# Autodesk Inventor assembly: Front_Panel_Assembly
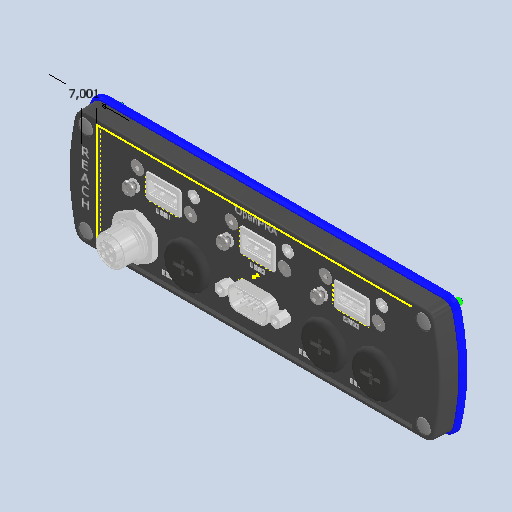
[picture p0: Inventor's stored thumbnail of the model, 512x512]
Saved by Autodesk Inventor 2022 (Build 260153000, 153)
## iProperties
Created: 2020-07-14
Part Number: Front_Panel_Assembly
Document SubType Name: Assembly
Designer: CASE-SMALL2
Author: CASE-SMALL2
## Documents named in this file (14)
- C:\Users\Viktor\Google Drive\Unicorn 2020\CAD_V2\Front_Panel\Front_Panel_Assembly.iam
- C:\Users\Viktor\Google Drive\Unicorn 2020\CAD_V2\Front_Panel\Panel\Front_Panel_Base_Assembly.iam
- C:\Users\Viktor\Google Drive\Unicorn 2020\CAD_V2\Front_Panel\Connectors\T4171110005-001\t4171110005-001.ipt
- C:\Users\Viktor\Google Drive\Unicorn 2020\CAD_V2\Front_Panel\Connectors\T4171110005-001\M12_NUT.ipt
- C:\Users\Viktor\Google Drive\Unicorn 2020\CAD_V2\Front_Panel\Connectors\MDBR-E09PM-JN0.ipt
- C:\Users\Viktor\Google Drive\Unicorn 2020\CAD_V2\Front_Panel\Connectors\MUSBR-3193-M0.ipt
- C:\Users\Viktor\Google Drive\Unicorn 2020\CAD_V2\Front_Panel\Connectors\MHDRA511M0.ipt
- C:\Users\Viktor\Google Drive\Unicorn 2020\CAD_V2\Front_Panel\Other\pop_PSZROX-0315.ipt
- C:\Users\Viktor\Google Drive\Unicorn 2020\CAD_V2\Front_Panel\Other\PG9x6mm_Plug.ipt
- C:\Users\Viktor\Google Drive\Unicorn 2020\CAD_V2\Front_Panel\Other\PG9x2.85mm_Nut.ipt
- C:\Users\Viktor\Google Drive\Unicorn 2020\CAD_V2\Front_Panel\Other\5207953-3.ipt
- C:\Users\Viktor\Google Drive\Unicorn 2020\CAD_V2\Front_Panel\Screws\ISO 4762 - M3 x 4ISO.ipt
- C:\Users\Viktor\Google Drive\Unicorn 2020\CAD_V2\Front_Panel\Screws\ISO 10642 - M3x6.ipt
- C:\Users\Viktor\Google Drive\Unicorn 2020\CAD_V2\Front_Panel\Screws\ISO 7380-1 - M3 x 8.ipt
## Components (37 placed, 13 different names)
1. Front_Pane_Basel_Assembly:1 [sub-assembly] — Rigid:1, Rigid:3, Rigid:7, Rigid:11, Rigid:17, Rigid:25, Rigid:36, Rigid:37, Rigid:38, Rigid:39, Rigid:42, Rigid:43, Rigid:45, Rigid:48, Rigid:47, Insert:1, Rigid:49, Rigid:50, Rigid:51, Rigid:52, Rigid:53, Rigid:54, Rigid:55, Rigid:56, Rigid:57, Rigid:58
2. t4171110005-001:1 — Rigid:45
3. M12_NUT:1 — Rigid:11
4. MDBR-E09PM-JN0:1 — Rigid:7
5. MUSBR-3193-M0:1 — Rigid:39
6. MUSBR-3193-M0:2 — Rigid:49
7. MUSBR-3193-M0:3 — Rigid:42, Rigid:44
8. MHDRA511M0:1 — Rigid:44
9. pop_PSZROX-0315:1 — Rigid:21, Rigid:32, Rigid:56
10. pop_PSZROX-0315:2 — Rigid:17, Rigid:20
11. pop_PSZROX-0315:3 — Rigid:22, Rigid:33, Rigid:55
12. pop_PSZROX-0315:4 — Rigid:23, Rigid:43
13. pop_PSZROX-0315:5 — Rigid:58, Rigid:59, Rigid:61
14. pop_PSZROX-0315:6 — Rigid:57, Rigid:60
15. PG9x6mm_Plug:1 — Rigid:1
16. PG9x6mm_Plug:2 — Insert:1, Angle:1
17. PG9x6mm_Plug:3 — Rigid:3, Angle:1
18. PG9x2.85mm_Nut:1 — Rigid:36
19. PG9x2.85mm_Nut:2 — Rigid:37
20. PG9x2.85mm_Nut:3 — Rigid:38
21. 5207953-3:1 — Rigid:48
22. 5207953-3:2 — Rigid:47
23. ISO 4762 - M3 x 4ISO:1 — Rigid:20
24. ISO 4762 - M3 x 4ISO:2 — Rigid:21
25. ISO 4762 - M3 x 4ISO:3 — Rigid:22
26. ISO 4762 - M3 x 4ISO:4 — Rigid:23
27. ISO 4762 - M3 x 4ISO:5 — Rigid:60
28. ISO 4762 - M3 x 4ISO:6 — Rigid:61
29. ISO 7380-1 - M3 x 8:3 — Rigid:32
30. ISO 7380-1 - M3 x 8:4 — Rigid:33
31. ISO 7380-1 - M3 x 8:5 — Rigid:59
32. ISO 10642 - M3x6:1 — Rigid:50
33. ISO 10642 - M3x6:2 — Rigid:25
34. ISO 10642 - M3x6:3 — Rigid:51
35. ISO 10642 - M3x6:4 — Rigid:52
36. ISO 10642 - M3x6:5 — Rigid:53
37. ISO 10642 - M3x6:6 — Rigid:54
## Relationships (37: WeldJoint 35, Insert 1, Angle 1)
- Rigid:1 [WeldJoint]: Front_Pane_Basel_Assembly:1 ↔ PG9x6mm_Plug:1
- Rigid:3 [WeldJoint]: Front_Pane_Basel_Assembly:1 ↔ PG9x6mm_Plug:3
- Rigid:7 [WeldJoint]: Front_Pane_Basel_Assembly:1 ↔ MDBR-E09PM-JN0:1
- Rigid:11 [WeldJoint]: Front_Pane_Basel_Assembly:1 ↔ M12_NUT:1
- Rigid:17 [WeldJoint]: Front_Pane_Basel_Assembly:1 ↔ pop_PSZROX-0315:2
- Rigid:20 [WeldJoint] (-2 mm): pop_PSZROX-0315:2 ↔ ISO 4762 - M3 x 4ISO:1
- Rigid:21 [WeldJoint] (-2 mm): pop_PSZROX-0315:1 ↔ ISO 4762 - M3 x 4ISO:2
- Rigid:22 [WeldJoint] (-2 mm): pop_PSZROX-0315:3 ↔ ISO 4762 - M3 x 4ISO:3
- Rigid:23 [WeldJoint] (-2 mm): pop_PSZROX-0315:4 ↔ ISO 4762 - M3 x 4ISO:4
- Rigid:25 [WeldJoint]: Front_Pane_Basel_Assembly:1 ↔ ISO 10642 - M3x6:2
- Rigid:32 [WeldJoint] (2 mm): pop_PSZROX-0315:1 ↔ ISO 7380-1 - M3 x 8:3
- Rigid:33 [WeldJoint] (2 mm): pop_PSZROX-0315:3 ↔ ISO 7380-1 - M3 x 8:4
- Rigid:36 [WeldJoint]: Front_Pane_Basel_Assembly:1 ↔ PG9x2.85mm_Nut:1
- Rigid:37 [WeldJoint]: Front_Pane_Basel_Assembly:1 ↔ PG9x2.85mm_Nut:2
- Rigid:38 [WeldJoint]: Front_Pane_Basel_Assembly:1 ↔ PG9x2.85mm_Nut:3
- Rigid:39 [WeldJoint]: Front_Pane_Basel_Assembly:1 ↔ MUSBR-3193-M0:1
- Rigid:42 [WeldJoint]: Front_Pane_Basel_Assembly:1 ↔ MUSBR-3193-M0:3
- Rigid:43 [WeldJoint]: Front_Pane_Basel_Assembly:1 ↔ pop_PSZROX-0315:4
- Rigid:44 [WeldJoint]: MUSBR-3193-M0:3 ↔ MHDRA511M0:1
- Rigid:45 [WeldJoint]: Front_Pane_Basel_Assembly:1 ↔ t4171110005-001:1
- Rigid:48 [WeldJoint]: Front_Pane_Basel_Assembly:1 ↔ 5207953-3:1
- Rigid:47 [WeldJoint]: Front_Pane_Basel_Assembly:1 ↔ 5207953-3:2
- Insert:1: Front_Pane_Basel_Assembly:1 ↔ PG9x6mm_Plug:2
- Angle:1 (0 deg): PG9x6mm_Plug:2 ↔ PG9x6mm_Plug:3
- Rigid:49 [WeldJoint]: Front_Pane_Basel_Assembly:1 ↔ MUSBR-3193-M0:2
- Rigid:50 [WeldJoint]: Front_Pane_Basel_Assembly:1 ↔ ISO 10642 - M3x6:1
- Rigid:51 [WeldJoint]: Front_Pane_Basel_Assembly:1 ↔ ISO 10642 - M3x6:3
- Rigid:52 [WeldJoint]: Front_Pane_Basel_Assembly:1 ↔ ISO 10642 - M3x6:4
- Rigid:53 [WeldJoint]: Front_Pane_Basel_Assembly:1 ↔ ISO 10642 - M3x6:5
- Rigid:54 [WeldJoint]: Front_Pane_Basel_Assembly:1 ↔ ISO 10642 - M3x6:6
- Rigid:55 [WeldJoint]: Front_Pane_Basel_Assembly:1 ↔ pop_PSZROX-0315:3
- Rigid:56 [WeldJoint]: Front_Pane_Basel_Assembly:1 ↔ pop_PSZROX-0315:1
- Rigid:57 [WeldJoint]: Front_Pane_Basel_Assembly:1 ↔ pop_PSZROX-0315:6
- Rigid:58 [WeldJoint]: Front_Pane_Basel_Assembly:1 ↔ pop_PSZROX-0315:5
- Rigid:59 [WeldJoint] (-2 mm): pop_PSZROX-0315:5 ↔ ISO 7380-1 - M3 x 8:5
- Rigid:60 [WeldJoint] (-2 mm): pop_PSZROX-0315:6 ↔ ISO 4762 - M3 x 4ISO:5
- Rigid:61 [WeldJoint] (2 mm): pop_PSZROX-0315:5 ↔ ISO 4762 - M3 x 4ISO:6
